# Autodesk Inventor assembly: SUBDriveTrainFrame
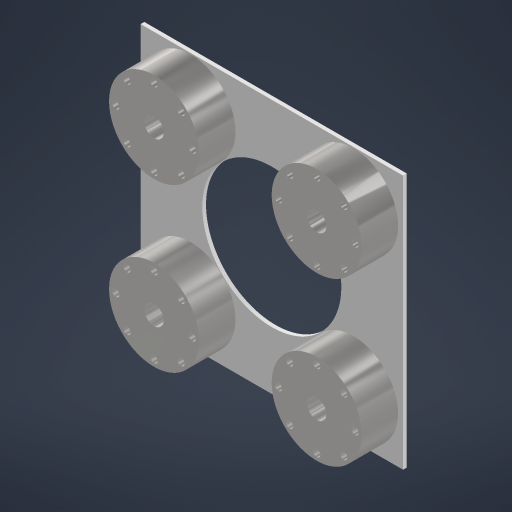
[picture p0: Inventor's stored thumbnail of the model, 512x512]
Saved by Autodesk Inventor 2024 (Build 280153000, 153)
## iProperties
Created: 2025-02-08
Part Number: SUBDriveTrainFrame
Document SubType Name: Assembly
Designer: Tommy Rohmann
Author: Tommy Rohmann
## Documents named in this file (4)
- C:\Users\Tommy Rohmann\OneDrive\Projects\Microgravity-Press-Washing-Machine\System Design and Documentation\Inventor Design Project\SUBDriveTrainFrame.iam
- C:\Users\Tommy Rohmann\OneDrive\Projects\Microgravity-Press-Washing-Machine\System Design and Documentation\Inventor Design Project\LAYOUT.ipt
- C:\Users\Tommy Rohmann\OneDrive\Projects\Microgravity-Press-Washing-Machine\System Design and Documentation\Inventor Design Project\LoadCellMountFrame.ipt
- C:\Users\Tommy Rohmann\OneDrive\Projects\Microgravity-Press-Washing-Machine\System Design and Documentation\Inventor Design Project\LoadCell.ipt
## Components (6 placed, 3 different names)
1. LAYOUT:1
2. LoadCellMountFrame:1 — Mate:1, Mate:2, Mate:3, Mate:4, Mate:5, Mate:6, Mate:7, Mate:8
3. LoadCell:1 — Mate:1, Mate:8
4. LoadCell:2 — Mate:2, Mate:7
5. LoadCell:3 — Mate:4, Mate:5
6. LoadCell:4 — Mate:3, Mate:6
## Relationships (9: Mate 8, Composite 1)
- [Composite]: LAYOUT:1 ↔ LoadCellMountFrame:1
- Mate:1: LoadCellMountFrame:1 ↔ LoadCell:1
- Mate:2: LoadCellMountFrame:1 ↔ LoadCell:2
- Mate:3: LoadCellMountFrame:1 ↔ LoadCell:4
- Mate:4: LoadCellMountFrame:1 ↔ LoadCell:3
- Mate:5: LoadCellMountFrame:1 ↔ LoadCell:3
- Mate:6: LoadCellMountFrame:1 ↔ LoadCell:4
- Mate:7: LoadCellMountFrame:1 ↔ LoadCell:2
- Mate:8: LoadCellMountFrame:1 ↔ LoadCell:1
